# Autodesk Inventor assembly: YawMotor
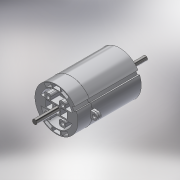
[picture p0: Inventor's stored thumbnail of the model, 180x180]
Saved by Autodesk Inventor 2018.2 (Build 222227000, 227)
## iProperties
Created: 2018-03-13
Part Number: YawMotor
Document SubType Name: Assembly
Designer: mansu
Sending System: SolidWorks 2017
Last Author: Wenoa
Last Saved: 2018-03-13
Author: mansu
## Documents named in this file (5)
- C:\Users\Moochster\OneDrive\Documents\2018 UBC\ELEC 391\Controller\cad\release\YawMotor.iam
- C:\Users\Moochster\OneDrive\Documents\2018 UBC\ELEC 391\Motor\SolidWorks\StatorShell_v3.ipt
- C:\Users\Moochster\OneDrive\Documents\2018 UBC\ELEC 391\Motor\SolidWorks\StatorShell_v3_attachment.ipt
- C:\Users\Moochster\OneDrive\Documents\2018 UBC\ELEC 391\Motor\SolidWorks\shaft_quarterinch.ipt
- C:\Users\Moochster\OneDrive\Documents\2018 UBC\ELEC 391\Motor\SolidWorks\pressurecap-back.ipt
## Components (4 placed, 4 different names)
1. StatorShell_v3:1 — Mate:1, Mate:2, Flush:1
2. StatorShell_v3_attachment:1 — Mate:1, Mate:2, Flush:1, Mate:3, Angle:1, Mate:6, Flush:2
3. shaft_quarterinch:1 — Mate:3, Mate:4, Flush:2
4. pressurecap-back:1 — Mate:4, Angle:1, Mate:6
## Relationships (8: Mate 5, Flush 2, Angle 1)
- Mate:1: StatorShell_v3:1 ↔ StatorShell_v3_attachment:1
- Mate:2 (0.1 mm): StatorShell_v3:1 ↔ StatorShell_v3_attachment:1
- Flush:1: StatorShell_v3:1 ↔ StatorShell_v3_attachment:1
- Mate:3: StatorShell_v3_attachment:1 ↔ shaft_quarterinch:1
- Mate:4: shaft_quarterinch:1 ↔ pressurecap-back:1
- Angle:1 (0 deg): StatorShell_v3_attachment:1 ↔ pressurecap-back:1
- Mate:6 (0.1 mm): StatorShell_v3_attachment:1 ↔ pressurecap-back:1
- Flush:2 (-30 mm): StatorShell_v3_attachment:1 ↔ shaft_quarterinch:1
